# Autodesk Inventor assembly: EnsambleCajaControl
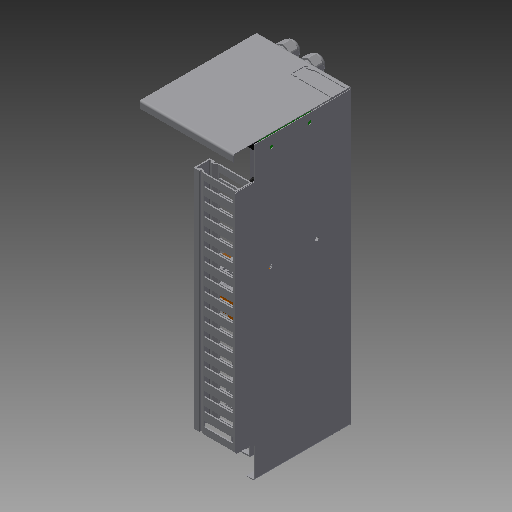
[picture p0: Inventor's stored thumbnail of the model, 512x512]
Saved by Autodesk Inventor 2017 (Build 210142000, 142)
## iProperties
Created: 2020-12-07
Part Number: EnsambleCajaControl
Document SubType Name: Assembly
Designer: USUARIO
Author: USUARIO
## Documents named in this file (14)
- D:\Laboratorio\Autoclave\Autoclave Horizontal\Sin Precamara\2020\Autoclave 23L con Vacio Health Import #004588445-46-47-48 OP2020363-364-365-366\Ensamble Caja Control\EnsambleCajaControl.iam
- D:\Laboratorio\Autoclave\Autoclave Horizontal\Sin Precamara\2020\Autoclave 23L con Vacio Health Import #004588445-46-47-48 OP2020363-364-365-366\Ensamble Caja Control\CAJA CONEXIONES ACH-23L-2020-V.ipt
- D:\Laboratorio\Autoclave\Autoclave Horizontal\Sin Precamara\2020\Autoclave 23L con Vacio Health Import #004588445-46-47-48 OP2020363-364-365-366\Schematic\Nextion Control SM\NextionControlV3.iam
- C:\Users\USUARIO\Documents\Inventor\Canaleta 30x60 450mm.iam
- C:\Users\USUARIO\Documents\Inventor\Canaleta 30x60 120mm.iam
- C:\Users\USUARIO\Documents\Inventor\Canaleta 30x60 348mm.iam
- C:\Modelos 3D y DXF\Ex9C 25-38-NOARK.stp\Ex9C 25-38-NOARK.ipt
- C:\Modelos 3D y DXF\B1A-NOARK.stp\75856.ipt
- C:\Modelos 3D y DXF\B1A-NOARK.stp\B1D 2P-NOARK.ipt
- C:\Modelos 3D y DXF\SSR\a24125pg.ipt
- C:\Users\USUARIO\Documents\Inventor\Canaleta 30x30 125mm.iam
- C:\Users\USUARIO\Documents\Inventor\Canaleta 40x40 80mm.iam
- C:\Modelos 3D y DXF\Prensacables\User Library-BUD CABLE GLAND.ipt
- C:\Users\USUARIO\Documents\Inventor\Riel170mm.ipt
## Components (16 placed, 13 different names)
1. CAJA CONEXIONES ACH-23L-2020-V:1 — Mate:1, Mate:2, Mate:3, Mate:4, Mate:5, Mate:7, Mate:10, Mate:11, Mate:12, Flush:1, Mate:13, Mate:15, Mate:17, Mate:19, Mate:20, Mate:21, Mate:23, Mate:25, Mate:26, Mate:27, Mate:30
2. NextionControlV3:1 [sub-assembly] — Mate:1, Mate:2, Mate:9
3. Canaleta 30x60 450mm:1 [sub-assembly] — Mate:3, Mate:4, Mate:5, Mate:8, Flush:2, Mate:14, Mate:16, Mate:22, Mate:24, Mate:29
4. Canaleta 30x60 120mm:1 [sub-assembly] — Mate:7, Mate:8, Mate:9, Mate:28
5. Canaleta 30x60 348mm:1 [sub-assembly] — Mate:10, Mate:11, Mate:12, Mate:18
6. Ex9C 25-38-NOARK:1 — Flush:1, Flush:2
7. 75856:1 — Mate:13, Mate:14
8. 75856:3 — Mate:15, Mate:16
9. B1D 2P-NOARK:1 — Mate:17, Mate:18
10. a24125pg:1 — Mate:19
11. a24125pg:3 — Mate:20, Mate:30
12. Canaleta 30x30 125mm:1 [sub-assembly] — Mate:21, Mate:22
13. Canaleta 40x40 80mm:1 [sub-assembly] — Mate:23, Mate:24
14. User Library-BUD CABLE GLAND:1 — Mate:25
15. User Library-BUD CABLE GLAND:2 — Mate:26
16. Riel170mm:1 — Mate:27, Mate:28, Mate:29
## Relationships (31: Mate 29, Flush 2)
- Mate:1 (13 mm): CAJA CONEXIONES ACH-23L-2020-V:1 ↔ NextionControlV3:1
- Mate:2 (10 mm): CAJA CONEXIONES ACH-23L-2020-V:1 ↔ NextionControlV3:1
- Mate:3: CAJA CONEXIONES ACH-23L-2020-V:1 ↔ Canaleta 30x60 450mm:1
- Mate:4 (5 mm): CAJA CONEXIONES ACH-23L-2020-V:1 ↔ Canaleta 30x60 450mm:1
- Mate:5: CAJA CONEXIONES ACH-23L-2020-V:1 ↔ Canaleta 30x60 450mm:1
- Mate:7: CAJA CONEXIONES ACH-23L-2020-V:1 ↔ Canaleta 30x60 120mm:1
- Mate:8: Canaleta 30x60 450mm:1 ↔ Canaleta 30x60 120mm:1
- Mate:9 (20 mm): NextionControlV3:1 ↔ Canaleta 30x60 120mm:1
- Mate:10: CAJA CONEXIONES ACH-23L-2020-V:1 ↔ Canaleta 30x60 348mm:1
- Mate:11 (2 mm): CAJA CONEXIONES ACH-23L-2020-V:1 ↔ Canaleta 30x60 348mm:1
- Mate:12 (-2 mm): CAJA CONEXIONES ACH-23L-2020-V:1 ↔ Canaleta 30x60 348mm:1
- Flush:1 (-2 mm): CAJA CONEXIONES ACH-23L-2020-V:1 ↔ Ex9C 25-38-NOARK:1
- Flush:2 (-15 mm): Canaleta 30x60 450mm:1 ↔ Ex9C 25-38-NOARK:1
- Mate:13 (3 mm): CAJA CONEXIONES ACH-23L-2020-V:1 ↔ 75856:1
- Mate:14 (15 mm): Canaleta 30x60 450mm:1 ↔ 75856:1
- Mate:15 (3 mm): CAJA CONEXIONES ACH-23L-2020-V:1 ↔ 75856:3
- Mate:16 (15 mm): Canaleta 30x60 450mm:1 ↔ 75856:3
- Mate:17 (3 mm): CAJA CONEXIONES ACH-23L-2020-V:1 ↔ B1D 2P-NOARK:1
- Mate:18 (15 mm): Canaleta 30x60 348mm:1 ↔ B1D 2P-NOARK:1
- Mate:19: CAJA CONEXIONES ACH-23L-2020-V:1 ↔ a24125pg:1
- Mate:20: CAJA CONEXIONES ACH-23L-2020-V:1 ↔ a24125pg:3
- Mate:21: CAJA CONEXIONES ACH-23L-2020-V:1 ↔ Canaleta 30x30 125mm:1
- Mate:22 (1 mm): Canaleta 30x60 450mm:1 ↔ Canaleta 30x30 125mm:1
- Mate:23: CAJA CONEXIONES ACH-23L-2020-V:1 ↔ Canaleta 40x40 80mm:1
- Mate:24: Canaleta 30x60 450mm:1 ↔ Canaleta 40x40 80mm:1
- Mate:25: CAJA CONEXIONES ACH-23L-2020-V:1 ↔ User Library-BUD CABLE GLAND:1
- Mate:26: CAJA CONEXIONES ACH-23L-2020-V:1 ↔ User Library-BUD CABLE GLAND:2
- Mate:27: CAJA CONEXIONES ACH-23L-2020-V:1 ↔ Riel170mm:1
- Mate:28: Canaleta 30x60 120mm:1 ↔ Riel170mm:1
- Mate:29 (45 mm): Canaleta 30x60 450mm:1 ↔ Riel170mm:1
- Mate:30 (80 mm): CAJA CONEXIONES ACH-23L-2020-V:1 ↔ a24125pg:3
